# Autodesk Inventor assembly: 153160 QSS-10
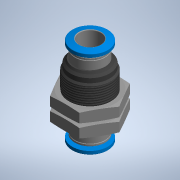
[picture p0: Inventor's stored thumbnail of the model, 180x180]
Saved by Autodesk Inventor 2021 (Build 250183000, 183)
## iProperties
Part Number: 153160 QSS-10
Catalog Web Link: www.cadenas.de
Description: QSS-Push-in bulkhead connector
Vendor: FESTO
Document SubType Name: Assembly
Designer: partserver
Manufacturer: FESTO
Mass: 35 g
Surface Area: 66.1971 cm^2
Volume: 9.28849 cm^3
Density: 3.7681 g/cm^3
Category: PARTsolutions
Company: FESTO
PSOL_IDENT_0: {ATYP=ASSISTANT},{DATA=script=$CADENAS_DATA/23d-libs/festo/webfesto.vbb/&M_FAMILY=QSS&M_GROUP=01&M_P
PSOL_IDENT_1: ARTNO=153160&IDCODE1=QSS-10&IDCODE2=&customer_number_cns=&MATES=1&LOD=HI&LOCKERP=0&SINGLEPART=1}
NB: 153160 QSS-10
NN: QSS
NT: Push-in bulkhead connector
NBSYN: $TNR. $TYP.
LINA: 153160 QSS-10
CATALOG: Festo
TNR: 153160
TYP: QSS-10
D1: 10
NENN: 9
D5: M20x1
D6: 18.5
L1: 42.4
L2: 21.6
L3: 11.9
L4: 5
SW: 24
T: 20.7
CNSMASSEXACT: 0.035
SUPPLIER: FESTO
ARTICLENO: 153160 QSS-10
BOMINFO: 153160 QSS-10
CREATOR: CADENAS GmbH
Title: 153160 QSS-10
Author: Cadenas PARTsolutions
Comments: Push-in bulkhead connector
## Documents named in this file (3)
- D:\Nelson\Documentos\Inventor\Proyecto_PAI\153160 QSS-10.iam
- D:\Nelson\Documentos\Inventor\Proyecto_PAI\153160 QSS-10---(part).ipt
- D:\Nelson\Documentos\Inventor\Proyecto_PAI\Flachmutter M20x1-5-24.ipt
## Components (3 placed, 2 different names)
1. 153160 QSS-10---(part):1 — IP1_XY@1 <-> SLE_XY@2, IP1_Z@1 <-> SLE_Z@2, IP1_YZ@1 <-> SLE_YZ@2, IP2_Z@1 <-> SLE_Z@3, IP2_YZ@1 <-> SLE_YZ@3
2. Flachmutter M20x1-5-24:1 — IP1_XY@1 <-> SLE_XY@2, IP1_Z@1 <-> SLE_Z@2, IP1_YZ@1 <-> SLE_YZ@2, Mate:4
3. Flachmutter M20x1-5-24:2 — IP2_Z@1 <-> SLE_Z@3, IP2_YZ@1 <-> SLE_YZ@3, Mate:4
## Relationships (6: Mate 3, Angle 2, Flush 1)
- IP1_XY@1 <-> SLE_XY@2 [Flush]: 153160 QSS-10---(part):1 ↔ Flachmutter M20x1-5-24:1
- IP1_Z@1 <-> SLE_Z@2 [Mate]: 153160 QSS-10---(part):1 ↔ Flachmutter M20x1-5-24:1
- IP1_YZ@1 <-> SLE_YZ@2 [Angle] (0 deg): 153160 QSS-10---(part):1 ↔ Flachmutter M20x1-5-24:1
- IP2_Z@1 <-> SLE_Z@3 [Mate]: 153160 QSS-10---(part):1 ↔ Flachmutter M20x1-5-24:2
- IP2_YZ@1 <-> SLE_YZ@3 [Angle] (0 deg): 153160 QSS-10---(part):1 ↔ Flachmutter M20x1-5-24:2
- Mate:4 (1.21 mm): Flachmutter M20x1-5-24:1 ↔ Flachmutter M20x1-5-24:2
